# Autodesk Inventor assembly: plugassmbly
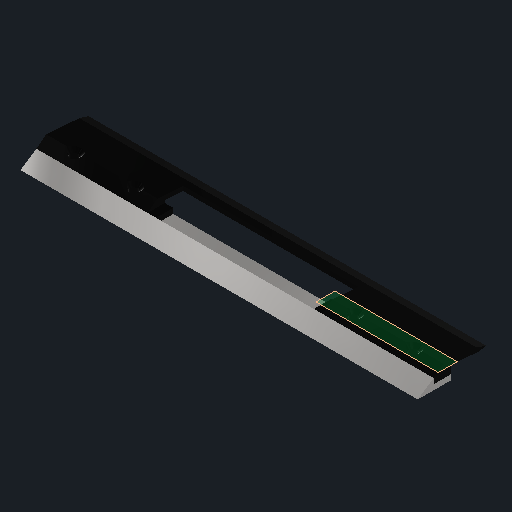
[picture p0: Inventor's stored thumbnail of the model, 512x512]
Saved by Autodesk Inventor 2026.2 (Build 302298010, 298A)
## iProperties
Created: 2026-05-09
Part Number: plugassmbly
Document SubType Name: Assembly
Designer: karol
Author: karol
## Documents named in this file (4)
- C:\Users\karol\Documents\GitHub\bolt\BOLT\cad\assembly\plugassmbly.iam
- C:\Users\karol\Documents\GitHub\bolt\BOLT\cad\ready parts\pługmoj.ipt
- C:\Users\karol\Documents\GitHub\bolt\BOLT\cad\ready parts\mocowanie do pługu.ipt
- C:\Users\karol\Documents\GitHub\bolt\BOLT\cad\ready parts\przódv3.ipt
## Components (3 placed, 3 different names)
1. pługmoj:1 — Zestawiające:1, Zestawiające:2, Zestawiające:3, Równoległe:1
2. mocowanie do pługu:1 — Zestawiające:1, Zestawiające:2, Zestawiające:3, Zestawiające:4, Równoległe:2
3. przódv3:1 — Zestawiające:4, Równoległe:1, Równoległe:2
## Relationships (6: Mate 4, Flush 2)
- Zestawiające:1 [Mate]: pługmoj:1 ↔ mocowanie do pługu:1
- Zestawiające:2 [Mate]: pługmoj:1 ↔ mocowanie do pługu:1
- Zestawiające:3 [Mate]: pługmoj:1 ↔ mocowanie do pługu:1
- Zestawiające:4 [Mate]: mocowanie do pługu:1 ↔ przódv3:1
- Równoległe:1 [Flush]: pługmoj:1 ↔ przódv3:1
- Równoległe:2 [Flush]: mocowanie do pługu:1 ↔ przódv3:1
